# Autodesk Inventor assembly: IntakeSlides4.0
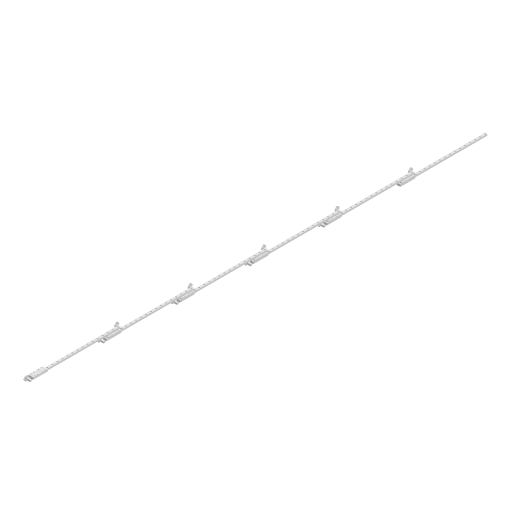
[picture p0: Inventor's stored thumbnail of the model, 512x512]
Saved by Autodesk Inventor 2023 (Build 270158000, 158)
## iProperties
Created: 2022-09-16
Part Number: IntakeSlides4.0
Document SubType Name: Assembly
Designer: deli
Author: deli
## Documents named in this file (7)
- C:\Users\deli\OneDrive - Eastside Preparatory School\FTC\8103-power-play\CAD\IntakeSlides4.0.iam
- C:\Users\deli\OneDrive - Eastside Preparatory School\FTC\8103-power-play\CAD\Carrige.ipt
- C:\Users\deli\OneDrive - Eastside Preparatory School\FTC\8103-power-play\CAD\Carrige Attatchment.ipt
- C:\Users\deli\OneDrive - Eastside Preparatory School\FTC\8103-power-play\CAD\FTC-parts\Mcmaster Carr\91294A126_Black-Oxide Alloy Steel Hex Drive Flat Head Screw.ipt
- C:\Users\deli\OneDrive - Eastside Preparatory School\FTC\8103-power-play\CAD\mgn9 350mm.ipt
- C:\Users\deli\OneDrive - Eastside Preparatory School\FTC\8103-power-play\CAD\mgn9SlideBearingHolder.ipt
- C:\Users\deli\OneDrive - Eastside Preparatory School\FTC\8103-power-play\CAD\Slides Bearings.iam
## Components (78 placed, 6 different names)
1. Carrige:3
2. Carrige:4 — Flush:21
3. Carrige Attatchment:2 — Mate:32, Mate:33, Angle:3, Mate:57, Mate:58, Mate:59
4. 91294A126_Black-Oxide Alloy Steel Hex Drive Flat Head Screw:9
5. 91294A126_Black-Oxide Alloy Steel Hex Drive Flat Head Screw:10
6. 91294A126_Black-Oxide Alloy Steel Hex Drive Flat Head Screw:11
7. 91294A126_Black-Oxide Alloy Steel Hex Drive Flat Head Screw:12
8. 91294A126_Black-Oxide Alloy Steel Hex Drive Flat Head Screw:13
9. 91294A126_Black-Oxide Alloy Steel Hex Drive Flat Head Screw:14
10. 91294A126_Black-Oxide Alloy Steel Hex Drive Flat Head Screw:15
11. 91294A126_Black-Oxide Alloy Steel Hex Drive Flat Head Screw:16
12. mgn9 350mm:2 — Flush:21
13. Slides Bearings:1 [sub-assembly] — Mate:32, Mate:33, Angle:3
14. Carrige:5
15. Carrige:6
16. Carrige Attatchment:3 — Mate:105, Mate:106, Mate:107
17. 91294A126_Black-Oxide Alloy Steel Hex Drive Flat Head Screw:17
18. 91294A126_Black-Oxide Alloy Steel Hex Drive Flat Head Screw:18
19. 91294A126_Black-Oxide Alloy Steel Hex Drive Flat Head Screw:19
20. 91294A126_Black-Oxide Alloy Steel Hex Drive Flat Head Screw:20
21. 91294A126_Black-Oxide Alloy Steel Hex Drive Flat Head Screw:21
22. 91294A126_Black-Oxide Alloy Steel Hex Drive Flat Head Screw:22
23. 91294A126_Black-Oxide Alloy Steel Hex Drive Flat Head Screw:23
24. 91294A126_Black-Oxide Alloy Steel Hex Drive Flat Head Screw:24
25. mgn9 350mm:3 — Mate:57, Mate:58, Mate:59
26. mgn9SlideBearingHolder:2
27. Slides Bearings:3 [sub-assembly]
28. Slides Bearings:4 [sub-assembly]
29. Carrige:7
30. Carrige:8
31. Carrige Attatchment:4
32. 91294A126_Black-Oxide Alloy Steel Hex Drive Flat Head Screw:25
33. 91294A126_Black-Oxide Alloy Steel Hex Drive Flat Head Screw:26
34. 91294A126_Black-Oxide Alloy Steel Hex Drive Flat Head Screw:27
35. 91294A126_Black-Oxide Alloy Steel Hex Drive Flat Head Screw:28
36. 91294A126_Black-Oxide Alloy Steel Hex Drive Flat Head Screw:29
37. 91294A126_Black-Oxide Alloy Steel Hex Drive Flat Head Screw:30
38. 91294A126_Black-Oxide Alloy Steel Hex Drive Flat Head Screw:31
39. 91294A126_Black-Oxide Alloy Steel Hex Drive Flat Head Screw:32
40. mgn9 350mm:4 — Mate:105, Mate:106, Mate:107
41. mgn9SlideBearingHolder:3
42. Slides Bearings:5 [sub-assembly]
43. Slides Bearings:6 [sub-assembly]
44. Carrige:9
45. Carrige:10
46. Carrige Attatchment:5 — Mate:153, Mate:154, Mate:155
47. 91294A126_Black-Oxide Alloy Steel Hex Drive Flat Head Screw:33
48. 91294A126_Black-Oxide Alloy Steel Hex Drive Flat Head Screw:34
49. 91294A126_Black-Oxide Alloy Steel Hex Drive Flat Head Screw:35
50. 91294A126_Black-Oxide Alloy Steel Hex Drive Flat Head Screw:36
51. 91294A126_Black-Oxide Alloy Steel Hex Drive Flat Head Screw:37
52. 91294A126_Black-Oxide Alloy Steel Hex Drive Flat Head Screw:38
53. 91294A126_Black-Oxide Alloy Steel Hex Drive Flat Head Screw:39
54. 91294A126_Black-Oxide Alloy Steel Hex Drive Flat Head Screw:40
55. mgn9 350mm:5
56. mgn9SlideBearingHolder:4
57. Slides Bearings:7 [sub-assembly]
58. Slides Bearings:8 [sub-assembly]
59. Carrige:11
60. Carrige:12
61. Carrige Attatchment:6
62. 91294A126_Black-Oxide Alloy Steel Hex Drive Flat Head Screw:41
63. 91294A126_Black-Oxide Alloy Steel Hex Drive Flat Head Screw:42
64. 91294A126_Black-Oxide Alloy Steel Hex Drive Flat Head Screw:43
65. 91294A126_Black-Oxide Alloy Steel Hex Drive Flat Head Screw:44
66. 91294A126_Black-Oxide Alloy Steel Hex Drive Flat Head Screw:45
67. 91294A126_Black-Oxide Alloy Steel Hex Drive Flat Head Screw:46
68. 91294A126_Black-Oxide Alloy Steel Hex Drive Flat Head Screw:47
69. 91294A126_Black-Oxide Alloy Steel Hex Drive Flat Head Screw:48
70. mgn9 350mm:6 — Mate:153, Mate:154, Mate:155
71. mgn9SlideBearingHolder:5
72. Slides Bearings:9 [sub-assembly]
73. Slides Bearings:10 [sub-assembly]
74. Carrige:13
75. Carrige:14
76. mgn9 350mm:7
77. mgn9SlideBearingHolder:6
78. Slides Bearings:12 [sub-assembly]
## Relationships (191: Mate 123, Flush 58, Angle 10)
- [Flush]: Carrige:3 ↔ Carrige:4
- [Flush]: Carrige:3 ↔ Carrige:4
- [Mate]: Carrige:3 ↔ Carrige:4
- [Mate]: Carrige:4 ↔ Carrige Attatchment:2
- [Mate]: Carrige:3 ↔ Carrige Attatchment:2
- [Mate]: Carrige:3 ↔ Carrige Attatchment:2
- [Mate]: Carrige Attatchment:2 ↔ 91294A126_Black-Oxide Alloy Steel Hex Drive Flat Head Screw:16
- [Mate]: Carrige Attatchment:2 ↔ 91294A126_Black-Oxide Alloy Steel Hex Drive Flat Head Screw:12
- [Mate]: Carrige Attatchment:2 ↔ 91294A126_Black-Oxide Alloy Steel Hex Drive Flat Head Screw:11
- [Mate]: Carrige Attatchment:2 ↔ 91294A126_Black-Oxide Alloy Steel Hex Drive Flat Head Screw:13
- [Mate]: Carrige Attatchment:2 ↔ 91294A126_Black-Oxide Alloy Steel Hex Drive Flat Head Screw:14
- [Mate]: Carrige Attatchment:2 ↔ 91294A126_Black-Oxide Alloy Steel Hex Drive Flat Head Screw:15
- [Mate]: Carrige Attatchment:2 ↔ 91294A126_Black-Oxide Alloy Steel Hex Drive Flat Head Screw:9
- [Mate]: Carrige Attatchment:2 ↔ 91294A126_Black-Oxide Alloy Steel Hex Drive Flat Head Screw:10
- [Flush]: Carrige Attatchment:2 ↔ 91294A126_Black-Oxide Alloy Steel Hex Drive Flat Head Screw:12
- [Flush]: Carrige Attatchment:2 ↔ 91294A126_Black-Oxide Alloy Steel Hex Drive Flat Head Screw:11
- [Flush]: Carrige Attatchment:2 ↔ 91294A126_Black-Oxide Alloy Steel Hex Drive Flat Head Screw:16
- [Flush]: Carrige Attatchment:2 ↔ 91294A126_Black-Oxide Alloy Steel Hex Drive Flat Head Screw:14
- [Flush]: Carrige Attatchment:2 ↔ 91294A126_Black-Oxide Alloy Steel Hex Drive Flat Head Screw:13
- [Flush]: Carrige Attatchment:2 ↔ 91294A126_Black-Oxide Alloy Steel Hex Drive Flat Head Screw:9
- [Flush]: Carrige Attatchment:2 ↔ 91294A126_Black-Oxide Alloy Steel Hex Drive Flat Head Screw:15
- [Flush]: Carrige Attatchment:2 ↔ 91294A126_Black-Oxide Alloy Steel Hex Drive Flat Head Screw:10
- [Mate]: Carrige:4 ↔ mgn9 350mm:2
- [Mate]: Carrige:4 ↔ mgn9 350mm:2
- Mate:32: Carrige Attatchment:2 ↔ Slides Bearings:1
- Mate:33: Carrige Attatchment:2 ↔ Slides Bearings:1
- Flush:21 (292.2 mm): Carrige:4 ↔ mgn9 350mm:2
- Angle:3 (45 deg): Carrige Attatchment:2 ↔ Slides Bearings:1
- [Flush]: Carrige:5 ↔ Carrige:6
- [Flush]: Carrige:5 ↔ Carrige:6
- [Mate]: Carrige:5 ↔ Carrige:6
- [Mate]: Carrige:6 ↔ Carrige Attatchment:3
- [Mate]: Carrige:5 ↔ Carrige Attatchment:3
- [Mate]: Carrige:5 ↔ Carrige Attatchment:3
- [Mate]: Carrige Attatchment:3 ↔ 91294A126_Black-Oxide Alloy Steel Hex Drive Flat Head Screw:24
- [Mate]: Carrige Attatchment:3 ↔ 91294A126_Black-Oxide Alloy Steel Hex Drive Flat Head Screw:20
- [Mate]: Carrige Attatchment:3 ↔ 91294A126_Black-Oxide Alloy Steel Hex Drive Flat Head Screw:19
- [Mate]: Carrige Attatchment:3 ↔ 91294A126_Black-Oxide Alloy Steel Hex Drive Flat Head Screw:21
- [Mate]: Carrige Attatchment:3 ↔ 91294A126_Black-Oxide Alloy Steel Hex Drive Flat Head Screw:22
- [Mate]: Carrige Attatchment:3 ↔ 91294A126_Black-Oxide Alloy Steel Hex Drive Flat Head Screw:23
- [Mate]: Carrige Attatchment:3 ↔ 91294A126_Black-Oxide Alloy Steel Hex Drive Flat Head Screw:17
- [Mate]: Carrige Attatchment:3 ↔ 91294A126_Black-Oxide Alloy Steel Hex Drive Flat Head Screw:18
- [Flush]: Carrige Attatchment:3 ↔ 91294A126_Black-Oxide Alloy Steel Hex Drive Flat Head Screw:20
- [Flush]: Carrige Attatchment:3 ↔ 91294A126_Black-Oxide Alloy Steel Hex Drive Flat Head Screw:19
- [Flush]: Carrige Attatchment:3 ↔ 91294A126_Black-Oxide Alloy Steel Hex Drive Flat Head Screw:24
- [Flush]: Carrige Attatchment:3 ↔ 91294A126_Black-Oxide Alloy Steel Hex Drive Flat Head Screw:22
- [Flush]: Carrige Attatchment:3 ↔ 91294A126_Black-Oxide Alloy Steel Hex Drive Flat Head Screw:21
- [Flush]: Carrige Attatchment:3 ↔ 91294A126_Black-Oxide Alloy Steel Hex Drive Flat Head Screw:17
- [Flush]: Carrige Attatchment:3 ↔ 91294A126_Black-Oxide Alloy Steel Hex Drive Flat Head Screw:23
- [Flush]: Carrige Attatchment:3 ↔ 91294A126_Black-Oxide Alloy Steel Hex Drive Flat Head Screw:18
- [Mate]: Carrige:6 ↔ mgn9 350mm:3
- [Mate]: Carrige:6 ↔ mgn9 350mm:3
- [Mate]: mgn9 350mm:3 ↔ mgn9SlideBearingHolder:2
- [Mate]: mgn9 350mm:3 ↔ mgn9SlideBearingHolder:2
- [Mate]: mgn9 350mm:3 ↔ mgn9SlideBearingHolder:2
- [Mate]: Carrige Attatchment:3 ↔ Slides Bearings:3
- [Mate]: Carrige Attatchment:3 ↔ Slides Bearings:3
- [Mate]: mgn9SlideBearingHolder:2 ↔ Slides Bearings:4
- [Mate]: mgn9SlideBearingHolder:2 ↔ Slides Bearings:4
- [Flush] (292.2 mm): Carrige:6 ↔ mgn9 350mm:3
- [Angle] (45 deg): Carrige Attatchment:3 ↔ Slides Bearings:3
- [Angle] (45 deg): mgn9SlideBearingHolder:2 ↔ Slides Bearings:4
- Mate:57: Carrige Attatchment:2 ↔ mgn9 350mm:3
- Mate:58: Carrige Attatchment:2 ↔ mgn9 350mm:3
- Mate:59: Carrige Attatchment:2 ↔ mgn9 350mm:3
- [Flush]: Carrige:7 ↔ Carrige:8
- [Flush]: Carrige:7 ↔ Carrige:8
- [Mate]: Carrige:7 ↔ Carrige:8
- [Mate]: Carrige:8 ↔ Carrige Attatchment:4
- [Mate]: Carrige:7 ↔ Carrige Attatchment:4
- [Mate]: Carrige:7 ↔ Carrige Attatchment:4
- [Mate]: Carrige Attatchment:4 ↔ 91294A126_Black-Oxide Alloy Steel Hex Drive Flat Head Screw:32
- [Mate]: Carrige Attatchment:4 ↔ 91294A126_Black-Oxide Alloy Steel Hex Drive Flat Head Screw:28
- [Mate]: Carrige Attatchment:4 ↔ 91294A126_Black-Oxide Alloy Steel Hex Drive Flat Head Screw:27
- [Mate]: Carrige Attatchment:4 ↔ 91294A126_Black-Oxide Alloy Steel Hex Drive Flat Head Screw:29
- [Mate]: Carrige Attatchment:4 ↔ 91294A126_Black-Oxide Alloy Steel Hex Drive Flat Head Screw:30
- [Mate]: Carrige Attatchment:4 ↔ 91294A126_Black-Oxide Alloy Steel Hex Drive Flat Head Screw:31
- [Mate]: Carrige Attatchment:4 ↔ 91294A126_Black-Oxide Alloy Steel Hex Drive Flat Head Screw:25
- [Mate]: Carrige Attatchment:4 ↔ 91294A126_Black-Oxide Alloy Steel Hex Drive Flat Head Screw:26
- [Flush]: Carrige Attatchment:4 ↔ 91294A126_Black-Oxide Alloy Steel Hex Drive Flat Head Screw:28
- [Flush]: Carrige Attatchment:4 ↔ 91294A126_Black-Oxide Alloy Steel Hex Drive Flat Head Screw:27
- [Flush]: Carrige Attatchment:4 ↔ 91294A126_Black-Oxide Alloy Steel Hex Drive Flat Head Screw:32
- [Flush]: Carrige Attatchment:4 ↔ 91294A126_Black-Oxide Alloy Steel Hex Drive Flat Head Screw:30
- [Flush]: Carrige Attatchment:4 ↔ 91294A126_Black-Oxide Alloy Steel Hex Drive Flat Head Screw:29
- [Flush]: Carrige Attatchment:4 ↔ 91294A126_Black-Oxide Alloy Steel Hex Drive Flat Head Screw:25
- [Flush]: Carrige Attatchment:4 ↔ 91294A126_Black-Oxide Alloy Steel Hex Drive Flat Head Screw:31
- [Flush]: Carrige Attatchment:4 ↔ 91294A126_Black-Oxide Alloy Steel Hex Drive Flat Head Screw:26
- [Mate]: Carrige:8 ↔ mgn9 350mm:4
- [Mate]: Carrige:8 ↔ mgn9 350mm:4
- [Mate]: mgn9 350mm:4 ↔ mgn9SlideBearingHolder:3
- [Mate]: mgn9 350mm:4 ↔ mgn9SlideBearingHolder:3
- [Mate]: mgn9 350mm:4 ↔ mgn9SlideBearingHolder:3
- [Mate]: Carrige Attatchment:4 ↔ Slides Bearings:5
- [Mate]: Carrige Attatchment:4 ↔ Slides Bearings:5
- [Mate]: mgn9SlideBearingHolder:3 ↔ Slides Bearings:6
- [Mate]: mgn9SlideBearingHolder:3 ↔ Slides Bearings:6
- [Flush] (292.2 mm): Carrige:8 ↔ mgn9 350mm:4
- [Angle] (45 deg): Carrige Attatchment:4 ↔ Slides Bearings:5
- [Angle] (45 deg): mgn9SlideBearingHolder:3 ↔ Slides Bearings:6
- [Flush]: Carrige:9 ↔ Carrige:10
- [Flush]: Carrige:9 ↔ Carrige:10
- [Mate]: Carrige:9 ↔ Carrige:10
- [Mate]: Carrige:10 ↔ Carrige Attatchment:5
- [Mate]: Carrige:9 ↔ Carrige Attatchment:5
- [Mate]: Carrige:9 ↔ Carrige Attatchment:5
- [Mate]: Carrige Attatchment:5 ↔ 91294A126_Black-Oxide Alloy Steel Hex Drive Flat Head Screw:40
- [Mate]: Carrige Attatchment:5 ↔ 91294A126_Black-Oxide Alloy Steel Hex Drive Flat Head Screw:36
- [Mate]: Carrige Attatchment:5 ↔ 91294A126_Black-Oxide Alloy Steel Hex Drive Flat Head Screw:35
- [Mate]: Carrige Attatchment:5 ↔ 91294A126_Black-Oxide Alloy Steel Hex Drive Flat Head Screw:37
- [Mate]: Carrige Attatchment:5 ↔ 91294A126_Black-Oxide Alloy Steel Hex Drive Flat Head Screw:38
- [Mate]: Carrige Attatchment:5 ↔ 91294A126_Black-Oxide Alloy Steel Hex Drive Flat Head Screw:39
- [Mate]: Carrige Attatchment:5 ↔ 91294A126_Black-Oxide Alloy Steel Hex Drive Flat Head Screw:33
- [Mate]: Carrige Attatchment:5 ↔ 91294A126_Black-Oxide Alloy Steel Hex Drive Flat Head Screw:34
- [Flush]: Carrige Attatchment:5 ↔ 91294A126_Black-Oxide Alloy Steel Hex Drive Flat Head Screw:36
- [Flush]: Carrige Attatchment:5 ↔ 91294A126_Black-Oxide Alloy Steel Hex Drive Flat Head Screw:35
- [Flush]: Carrige Attatchment:5 ↔ 91294A126_Black-Oxide Alloy Steel Hex Drive Flat Head Screw:40
- [Flush]: Carrige Attatchment:5 ↔ 91294A126_Black-Oxide Alloy Steel Hex Drive Flat Head Screw:38
- [Flush]: Carrige Attatchment:5 ↔ 91294A126_Black-Oxide Alloy Steel Hex Drive Flat Head Screw:37
- [Flush]: Carrige Attatchment:5 ↔ 91294A126_Black-Oxide Alloy Steel Hex Drive Flat Head Screw:33
- [Flush]: Carrige Attatchment:5 ↔ 91294A126_Black-Oxide Alloy Steel Hex Drive Flat Head Screw:39
- [Flush]: Carrige Attatchment:5 ↔ 91294A126_Black-Oxide Alloy Steel Hex Drive Flat Head Screw:34
- [Mate]: Carrige:10 ↔ mgn9 350mm:5
- [Mate]: Carrige:10 ↔ mgn9 350mm:5
- [Mate]: mgn9 350mm:5 ↔ mgn9SlideBearingHolder:4
- [Mate]: mgn9 350mm:5 ↔ mgn9SlideBearingHolder:4
- [Mate]: mgn9 350mm:5 ↔ mgn9SlideBearingHolder:4
- [Mate]: Carrige Attatchment:5 ↔ Slides Bearings:7
- [Mate]: Carrige Attatchment:5 ↔ Slides Bearings:7
- [Mate]: mgn9SlideBearingHolder:4 ↔ Slides Bearings:8
- [Mate]: mgn9SlideBearingHolder:4 ↔ Slides Bearings:8
- [Flush] (292.2 mm): Carrige:10 ↔ mgn9 350mm:5
- [Angle] (45 deg): Carrige Attatchment:5 ↔ Slides Bearings:7
- [Angle] (45 deg): mgn9SlideBearingHolder:4 ↔ Slides Bearings:8
- [Mate]: Carrige Attatchment:4 ↔ mgn9 350mm:5
- [Mate]: Carrige Attatchment:4 ↔ mgn9 350mm:5
- [Mate]: Carrige Attatchment:4 ↔ mgn9 350mm:5
- Mate:105: Carrige Attatchment:3 ↔ mgn9 350mm:4
- Mate:106: Carrige Attatchment:3 ↔ mgn9 350mm:4
- Mate:107: Carrige Attatchment:3 ↔ mgn9 350mm:4
- [Flush]: Carrige:11 ↔ Carrige:12
- [Flush]: Carrige:11 ↔ Carrige:12
- [Mate]: Carrige:11 ↔ Carrige:12
- [Mate]: Carrige:12 ↔ Carrige Attatchment:6
- [Mate]: Carrige:11 ↔ Carrige Attatchment:6
- [Mate]: Carrige:11 ↔ Carrige Attatchment:6
- [Mate]: Carrige Attatchment:6 ↔ 91294A126_Black-Oxide Alloy Steel Hex Drive Flat Head Screw:48
- [Mate]: Carrige Attatchment:6 ↔ 91294A126_Black-Oxide Alloy Steel Hex Drive Flat Head Screw:44
- [Mate]: Carrige Attatchment:6 ↔ 91294A126_Black-Oxide Alloy Steel Hex Drive Flat Head Screw:43
- [Mate]: Carrige Attatchment:6 ↔ 91294A126_Black-Oxide Alloy Steel Hex Drive Flat Head Screw:45
- [Mate]: Carrige Attatchment:6 ↔ 91294A126_Black-Oxide Alloy Steel Hex Drive Flat Head Screw:46
- [Mate]: Carrige Attatchment:6 ↔ 91294A126_Black-Oxide Alloy Steel Hex Drive Flat Head Screw:47
- [Mate]: Carrige Attatchment:6 ↔ 91294A126_Black-Oxide Alloy Steel Hex Drive Flat Head Screw:41
- [Mate]: Carrige Attatchment:6 ↔ 91294A126_Black-Oxide Alloy Steel Hex Drive Flat Head Screw:42
- [Flush]: Carrige Attatchment:6 ↔ 91294A126_Black-Oxide Alloy Steel Hex Drive Flat Head Screw:44
- [Flush]: Carrige Attatchment:6 ↔ 91294A126_Black-Oxide Alloy Steel Hex Drive Flat Head Screw:43
- [Flush]: Carrige Attatchment:6 ↔ 91294A126_Black-Oxide Alloy Steel Hex Drive Flat Head Screw:48
- [Flush]: Carrige Attatchment:6 ↔ 91294A126_Black-Oxide Alloy Steel Hex Drive Flat Head Screw:46
- [Flush]: Carrige Attatchment:6 ↔ 91294A126_Black-Oxide Alloy Steel Hex Drive Flat Head Screw:45
- [Flush]: Carrige Attatchment:6 ↔ 91294A126_Black-Oxide Alloy Steel Hex Drive Flat Head Screw:41
- [Flush]: Carrige Attatchment:6 ↔ 91294A126_Black-Oxide Alloy Steel Hex Drive Flat Head Screw:47
- [Flush]: Carrige Attatchment:6 ↔ 91294A126_Black-Oxide Alloy Steel Hex Drive Flat Head Screw:42
- [Mate]: Carrige:12 ↔ mgn9 350mm:6
- [Mate]: Carrige:12 ↔ mgn9 350mm:6
- [Mate]: mgn9 350mm:6 ↔ mgn9SlideBearingHolder:5
- [Mate]: mgn9 350mm:6 ↔ mgn9SlideBearingHolder:5
- [Mate]: mgn9 350mm:6 ↔ mgn9SlideBearingHolder:5
- [Mate]: Carrige Attatchment:6 ↔ Slides Bearings:9
- [Mate]: Carrige Attatchment:6 ↔ Slides Bearings:9
- [Mate]: mgn9SlideBearingHolder:5 ↔ Slides Bearings:10
- [Mate]: mgn9SlideBearingHolder:5 ↔ Slides Bearings:10
- [Flush] (292.2 mm): Carrige:12 ↔ mgn9 350mm:6
- [Angle] (45 deg): Carrige Attatchment:6 ↔ Slides Bearings:9
- [Angle] (45 deg): mgn9SlideBearingHolder:5 ↔ Slides Bearings:10
- [Flush]: Carrige:13 ↔ Carrige:14
- [Flush]: Carrige:13 ↔ Carrige:14
- [Mate]: Carrige:13 ↔ Carrige:14
- [Mate]: Carrige:14 ↔ mgn9 350mm:7
- [Mate]: Carrige:14 ↔ mgn9 350mm:7
- [Mate]: mgn9 350mm:7 ↔ mgn9SlideBearingHolder:6
- [Mate]: mgn9 350mm:7 ↔ mgn9SlideBearingHolder:6
- [Mate]: mgn9 350mm:7 ↔ mgn9SlideBearingHolder:6
- [Mate]: mgn9SlideBearingHolder:6 ↔ Slides Bearings:12
- [Mate]: mgn9SlideBearingHolder:6 ↔ Slides Bearings:12
- [Flush] (292.2 mm): Carrige:14 ↔ mgn9 350mm:7
- [Angle] (45 deg): mgn9SlideBearingHolder:6 ↔ Slides Bearings:12
- [Mate]: Carrige Attatchment:6 ↔ mgn9 350mm:7
- [Mate]: Carrige Attatchment:6 ↔ mgn9 350mm:7
- [Mate]: Carrige Attatchment:6 ↔ mgn9 350mm:7
- Mate:153: Carrige Attatchment:5 ↔ mgn9 350mm:6
- Mate:154: Carrige Attatchment:5 ↔ mgn9 350mm:6
- Mate:155: Carrige Attatchment:5 ↔ mgn9 350mm:6
## Named parameters: stroke = 292.2 mm, d170_d117 = 0 mm, d171_d118 = 0 mm, d172_d119 = 0 mm, d173_d122 = 0 mm, d174_d127 = 0 mm, d175_d128 = 0 mm, d176_d132 = 0 mm, d177_d133 = 0 mm, d178_d134 = 0 mm, d179_d135 = 0 mm, d180_d136 = 0 mm, d181_d137 = 0 mm, d182_d138 = 0 mm, d183_d139 = 0 mm, d184_d140 = 0 mm, d185_d141 = 0 mm, d186_d142 = 0 mm, d187_d143 = 0 mm, d188_d144 = 0 mm, d189_d145 = 0 mm, d190_d146 = 0 mm, d191_d147 = 0 mm, d192_d148 = 0 mm, d333_stroke = 292.2 mm, d334_d149 = 0 mm, d335_d150 = 0 mm, d336_d151 = 0 mm, d337_d152 = 0 mm, d338_d170_d117 = 0 mm, d339_d171_d118 = 0 mm, d340_d172_d119 = 0 mm, d341_d173_d122 = 0 mm, d342_d174_d127 = 0 mm, d343_d175_d128 = 0 mm, d344_d176_d132 = 0 mm, d345_d177_d133 = 0 mm, d346_d178_d134 = 0 mm, d347_d179_d135 = 0 mm, d348_d180_d136 = 0 mm, d349_d181_d137 = 0 mm, d350_d182_d138 = 0 mm, d351_d183_d139 = 0 mm, d352_d184_d140 = 0 mm, d353_d185_d141 = 0 mm, d354_d186_d142 = 0 mm, d355_d187_d143 = 0 mm, d356_d188_d144 = 0 mm, d357_d189_d145 = 0 mm, d358_d190_d146 = 0 mm, d359_d191_d147 = 0 mm, d360_d192_d148 = 0 mm, d361_d324 = 0 mm, d362_d325 = 0 mm, d363_d327 = 0 mm, d364_d328 = 0 mm, d365_d330 = 292.2 mm, d366_d331 = 45 deg, d367_d332 = 45 deg, d371_stroke = 292.2 mm, d372_d149 = 0 mm, d373_d150 = 0 mm, d374_d151 = 0 mm, d375_d152 = 0 mm, d376_d170_d117 = 0 mm, d377_d171_d118 = 0 mm, d378_d172_d119 = 0 mm, d379_d173_d122 = 0 mm, d380_d174_d127 = 0 mm, d381_d175_d128 = 0 mm, d382_d176_d132 = 0 mm, d383_d177_d133 = 0 mm, d384_d178_d134 = 0 mm, d385_d179_d135 = 0 mm, d386_d180_d136 = 0 mm, d387_d181_d137 = 0 mm, d388_d182_d138 = 0 mm, d389_d183_d139 = 0 mm, d390_d184_d140 = 0 mm, d391_d185_d141 = 0 mm, d392_d186_d142 = 0 mm, d393_d187_d143 = 0 mm, d394_d188_d144 = 0 mm, d395_d189_d145 = 0 mm, d396_d190_d146 = 0 mm, d397_d191_d147 = 0 mm, d398_d192_d148 = 0 mm, d399_d324 = 0 mm, d400_d325 = 0 mm, d401_d327 = 0 mm, d402_d328 = 0 mm, d403_d330 = 292.2 mm, d404_d331 = 45 deg, d405_d332 = 45 deg, d406_d333_stroke = 292.2 mm, d407_d334_d149 = 0 mm, d408_d335_d150 = 0 mm, d409_d336_d151 = 0 mm, d410_d337_d152 = 0 mm, d411_d338_d170_d117 = 0 mm, d412_d339_d171_d118 = 0 mm, d413_d340_d172_d119 = 0 mm, d414_d341_d173_d122 = 0 mm, d415_d342_d174_d127 = 0 mm, d416_d343_d175_d128 = 0 mm, d417_d344_d176_d132 = 0 mm, d418_d345_d177_d133 = 0 mm, d419_d346_d178_d134 = 0 mm, d420_d347_d179_d135 = 0 mm, d421_d348_d180_d136 = 0 mm, d422_d349_d181_d137 = 0 mm, d423_d350_d182_d138 = 0 mm, d424_d351_d183_d139 = 0 mm, d425_d352_d184_d140 = 0 mm, d426_d353_d185_d141 = 0 mm, d427_d354_d186_d142 = 0 mm, d428_d355_d187_d143 = 0 mm, d429_d356_d188_d144 = 0 mm, d430_d357_d189_d145 = 0 mm, d431_d358_d190_d146 = 0 mm, d432_d359_d191_d147 = 0 mm, d433_d360_d192_d148 = 0 mm, d434_d361_d324 = 0 mm, d435_d362_d325 = 0 mm, d436_d363_d327 = 0 mm, d437_d364_d328 = 0 mm, d438_d365_d330 = 292.2 mm, d439_d366_d331 = 45 deg, d440_d367_d332 = 45 deg, d441_d368 = 0 mm, d442_d369 = 0 mm, d443_d370 = 0 mm, d447_stroke = 292.2 mm, d448_d149 = 0 mm, d449_d150 = 0 mm, d450_d151 = 0 mm, d451_d152 = 0 mm, d452_d170_d117 = 0 mm, d453_d171_d118 = 0 mm, d454_d172_d119 = 0 mm, d455_d173_d122 = 0 mm, d456_d174_d127 = 0 mm, d457_d175_d128 = 0 mm, d458_d176_d132 = 0 mm, d459_d177_d133 = 0 mm, d460_d178_d134 = 0 mm, d461_d179_d135 = 0 mm, d462_d180_d136 = 0 mm, d463_d181_d137 = 0 mm, d464_d182_d138 = 0 mm, d465_d183_d139 = 0 mm, d466_d184_d140 = 0 mm, d467_d185_d141 = 0 mm, d468_d186_d142 = 0 mm, d469_d187_d143 = 0 mm, d470_d188_d144 = 0 mm, d471_d189_d145 = 0 mm, d472_d190_d146 = 0 mm, d473_d191_d147 = 0 mm, d474_d192_d148 = 0 mm, d475_d324 = 0 mm, d476_d325 = 0 mm, d477_d327 = 0 mm, d478_d328 = 0 mm, d479_d330 = 292.2 mm, d480_d331 = 45 deg, d481_d332 = 45 deg, d482_d333_stroke = 292.2 mm, d483_d334_d149 = 0 mm, d484_d335_d150 = 0 mm, d485_d336_d151 = 0 mm, d486_d337_d152 = 0 mm, d487_d338_d170_d117 = 0 mm, d488_d339_d171_d118 = 0 mm, d489_d340_d172_d119 = 0 mm, d509_d360_d192_d148 = 0 mm, d512_d363_d327 = 0 mm, d513_d364_d328 = 0 mm, d514_d365_d330 = 292.2 mm, d516_d367_d332 = 45 deg, d517_d368 = 0 mm, d518_d369 = 0 mm, d519_d370 = 0 mm
